# Autodesk Inventor assembly: X_galvo_Newport_assembly
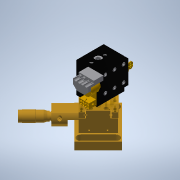
[picture p0: Inventor's stored thumbnail of the model, 180x180]
Saved by Autodesk Inventor 2022 (Build 260153000, 153)
## iProperties
Created: 2018-06-13
Part Number: X_galvo_Newport_assembly
Document SubType Name: Assembly
Designer: legant_local
Author: legant_local
## Documents named in this file (12)
- G:\My Drive\OPM\2P-OPM_CAD\workspace\Sub-assemblies\X_galvo_Newport_assembly.iam
- G:\My Drive\OPM\2P-OPM_CAD\workspace\Imported Components\Cambridge_Technology\D05893 w_D07861.ipt
- G:\My Drive\OPM\2P-OPM_CAD\workspace\Imported Components\McMaster_Carr\McMaster_Carr_91292A014_M2p5x10mm_socket_cap.ipt
- G:\My Drive\OPM\2P-OPM_CAD\workspace\Imported Components\McMaster_Carr\McMaster_Carr_92290A746_M2x16mm_socket_cap.ipt
- G:\My Drive\OPM\2P-OPM_CAD\workspace\Custom Parts Linked With Drawings\xgalvo_to_base_clamp.ipt
- G:\My Drive\OPM\2P-OPM_CAD\workspace\Custom 3D Printed Parts\galvo_stop.ipt
- G:\My Drive\OPM\2P-OPM_CAD\workspace\Custom 3D Printed Parts\zgalvo_cover.ipt
- G:\My Drive\OPM\2P-OPM_CAD\workspace\Custom Parts Linked With Drawings\xgalvo_to_newport_stage.ipt
- G:\My Drive\OPM\2P-OPM_CAD\workspace\Imported Components\Newport\Newport-9066-XY.ipt
- G:\My Drive\OPM\2P-OPM_CAD\workspace\Imported Components\Newport\Newport-SM-13.ipt
- G:\My Drive\OPM\2P-OPM_CAD\workspace\Imported Components\McMaster_Carr\McMaster_Carr_92185A203_8-32x1.5in_socket_cap.ipt
- G:\My Drive\OPM\2P-OPM_CAD\workspace\Imported Components\McMaster_Carr\McMaster_Carr_92185A546_0.25in-20x1.5in_socket_cap.ipt
## Components (19 placed, 11 different names)
1. D05893 w_D07861:1 — Mate:1, Angle:1
2. xgalvo_to_newport_stage:1 — Mate:1, Angle:1, Flush:12, Mate:39, Mate:40, Mate:55, Mate:56, Angle:72, Mate:66, Mate:67, Angle:73, Mate:72, Mate:73, Mate:74, Mate:75, Mate:76, Mate:77
3. McMaster_Carr_91292A014_M2p5x10mm_socket_cap:1 — Flush:4, Flush:5, Mate:13, Mate:16, Flush:13, Flush:14, Flush:15
4. McMaster_Carr_91292A014_M2p5x10mm_socket_cap:2 — Flush:4, Mate:14
5. McMaster_Carr_91292A014_M2p5x10mm_socket_cap:3 — Flush:5, Mate:15
6. xgalvo_to_base_clamp:1 — Flush:12, Mate:13, Mate:14, Mate:15, Mate:28, Mate:29, Mate:30, Mate:16, Mate:40, Angle:73
7. McMaster_Carr_91292A014_M2p5x10mm_socket_cap:4 — Flush:13, Mate:28
8. McMaster_Carr_91292A014_M2p5x10mm_socket_cap:5 — Flush:14, Mate:29
9. McMaster_Carr_91292A014_M2p5x10mm_socket_cap:6 — Flush:15, Mate:30
10. galvo_stop:1 — Mate:39, Mate:54, Mate:55, Mate:56, Mate:57, Mate:58
11. McMaster_Carr_92290A746_M2x16mm_socket_cap:1 — Mate:54, Mate:57
12. McMaster_Carr_92290A746_M2x16mm_socket_cap:2 — Mate:58
13. zgalvo_cover:1
14. Newport-9066-XY:1 — Angle:72, Mate:66, Mate:67, Mate:68, Mate:69
15. Newport-SM-13:1 — Mate:68
16. Newport-SM-13:2 — Mate:69
17. McMaster_Carr_92185A203_8-32x1.5in_socket_cap:1 — Mate:73, Mate:75
18. McMaster_Carr_92185A203_8-32x1.5in_socket_cap:2 — Mate:72, Mate:74
19. McMaster_Carr_92185A546_0.25in-20x1.5in_socket_cap:1 — Mate:76, Mate:77
## Relationships (35: Mate 26, Flush 6, Angle 3)
- Mate:1: D05893 w_D07861:1 ↔ xgalvo_to_newport_stage:1
- Angle:1 (225 deg): D05893 w_D07861:1 ↔ xgalvo_to_newport_stage:1
- Flush:4: McMaster_Carr_91292A014_M2p5x10mm_socket_cap:1 ↔ McMaster_Carr_91292A014_M2p5x10mm_socket_cap:2
- Flush:5: McMaster_Carr_91292A014_M2p5x10mm_socket_cap:1 ↔ McMaster_Carr_91292A014_M2p5x10mm_socket_cap:3
- Mate:13: McMaster_Carr_91292A014_M2p5x10mm_socket_cap:1 ↔ xgalvo_to_base_clamp:1
- Mate:14: McMaster_Carr_91292A014_M2p5x10mm_socket_cap:2 ↔ xgalvo_to_base_clamp:1
- Mate:15: McMaster_Carr_91292A014_M2p5x10mm_socket_cap:3 ↔ xgalvo_to_base_clamp:1
- Mate:16: McMaster_Carr_91292A014_M2p5x10mm_socket_cap:1 ↔ xgalvo_to_base_clamp:1
- Flush:12: xgalvo_to_newport_stage:1 ↔ xgalvo_to_base_clamp:1
- Flush:13: McMaster_Carr_91292A014_M2p5x10mm_socket_cap:1 ↔ McMaster_Carr_91292A014_M2p5x10mm_socket_cap:4
- Flush:14: McMaster_Carr_91292A014_M2p5x10mm_socket_cap:1 ↔ McMaster_Carr_91292A014_M2p5x10mm_socket_cap:5
- Flush:15: McMaster_Carr_91292A014_M2p5x10mm_socket_cap:1 ↔ McMaster_Carr_91292A014_M2p5x10mm_socket_cap:6
- Mate:28: xgalvo_to_base_clamp:1 ↔ McMaster_Carr_91292A014_M2p5x10mm_socket_cap:4
- Mate:29: xgalvo_to_base_clamp:1 ↔ McMaster_Carr_91292A014_M2p5x10mm_socket_cap:5
- Mate:30: xgalvo_to_base_clamp:1 ↔ McMaster_Carr_91292A014_M2p5x10mm_socket_cap:6
- [Mate]: galvo_stop:1 ↔ McMaster_Carr_92290A746_M2x16mm_socket_cap:2
- Mate:39: xgalvo_to_newport_stage:1 ↔ galvo_stop:1
- Mate:40: xgalvo_to_newport_stage:1 ↔ xgalvo_to_base_clamp:1
- Mate:54: galvo_stop:1 ↔ McMaster_Carr_92290A746_M2x16mm_socket_cap:1
- Mate:55: xgalvo_to_newport_stage:1 ↔ galvo_stop:1
- Mate:56: xgalvo_to_newport_stage:1 ↔ galvo_stop:1
- Mate:57: galvo_stop:1 ↔ McMaster_Carr_92290A746_M2x16mm_socket_cap:1
- Mate:58: galvo_stop:1 ↔ McMaster_Carr_92290A746_M2x16mm_socket_cap:2
- Angle:72 (0 deg): xgalvo_to_newport_stage:1 ↔ Newport-9066-XY:1
- Mate:66: xgalvo_to_newport_stage:1 ↔ Newport-9066-XY:1
- Mate:67: xgalvo_to_newport_stage:1 ↔ Newport-9066-XY:1
- Mate:68: Newport-9066-XY:1 ↔ Newport-SM-13:1
- Mate:69: Newport-9066-XY:1 ↔ Newport-SM-13:2
- Angle:73 (0 deg): xgalvo_to_newport_stage:1 ↔ xgalvo_to_base_clamp:1
- Mate:72: xgalvo_to_newport_stage:1 ↔ McMaster_Carr_92185A203_8-32x1.5in_socket_cap:2
- Mate:73: xgalvo_to_newport_stage:1 ↔ McMaster_Carr_92185A203_8-32x1.5in_socket_cap:1
- Mate:74: xgalvo_to_newport_stage:1 ↔ McMaster_Carr_92185A203_8-32x1.5in_socket_cap:2
- Mate:75: xgalvo_to_newport_stage:1 ↔ McMaster_Carr_92185A203_8-32x1.5in_socket_cap:1
- Mate:76: xgalvo_to_newport_stage:1 ↔ McMaster_Carr_92185A546_0.25in-20x1.5in_socket_cap:1
- Mate:77: xgalvo_to_newport_stage:1 ↔ McMaster_Carr_92185A546_0.25in-20x1.5in_socket_cap:1
## Named parameters: d61_d34 = 0 mm
